# Autodesk Inventor assembly: AX-12A
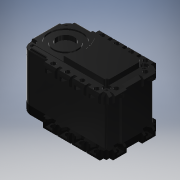
[picture p0: Inventor's stored thumbnail of the model, 180x180]
Saved by Autodesk Inventor 2019 (Build 230136000, 136)
## iProperties
Created: 2017-02-26
Part Number: AX-12A
Material: Типовые
Document SubType Name: Assembly
Designer: sbnnl
Author: sbnnl
Revision Number: ANY
## Documents named in this file (4)
- E:\IVAN\Ivan_desktop\Kvantorium\Competitions\INOP_2020\hardware\SCARA(Dynamixels)\components\Сервомотор Dynamixel AX-12-A\AX-12A.iam
- E:\IVAN\Ivan_desktop\Kvantorium\Competitions\INOP_2020\hardware\SCARA(Dynamixels)\components\Сервомотор Dynamixel AX-12-A\AX-12A-01.ipt
- E:\IVAN\Ivan_desktop\Kvantorium\Competitions\INOP_2020\hardware\SCARA(Dynamixels)\components\Сервомотор Dynamixel AX-12-A\AX-12A-02.ipt
- E:\IVAN\Ivan_desktop\Kvantorium\Competitions\INOP_2020\hardware\SCARA(Dynamixels)\components\Сервомотор Dynamixel AX-12-A\AX-12A-03.ipt
## Components (3 placed, 3 different names)
1. AX-12A-01_41 — Совмещение:3, Заподлицо:1, Заподлицо:2, Заподлицо:3, Заподлицо:4, Совмещение:4
2. AX-12A-02_42 — Заподлицо:3, Заподлицо:4, Совмещение:4
3. AX-12A-03_43 — Совмещение:3, Заподлицо:1, Заподлицо:2
## Relationships (6: Flush 4, Mate 2)
- Совмещение:3 [Mate]: AX-12A-01_41 ↔ AX-12A-03_43
- Заподлицо:1 [Flush]: AX-12A-01_41 ↔ AX-12A-03_43
- Заподлицо:2 [Flush]: AX-12A-01_41 ↔ AX-12A-03_43
- Заподлицо:3 [Flush]: AX-12A-01_41 ↔ AX-12A-02_42
- Заподлицо:4 [Flush]: AX-12A-01_41 ↔ AX-12A-02_42
- Совмещение:4 [Mate]: AX-12A-01_41 ↔ AX-12A-02_42
